# Autodesk Inventor assembly: Assembly Rack_4
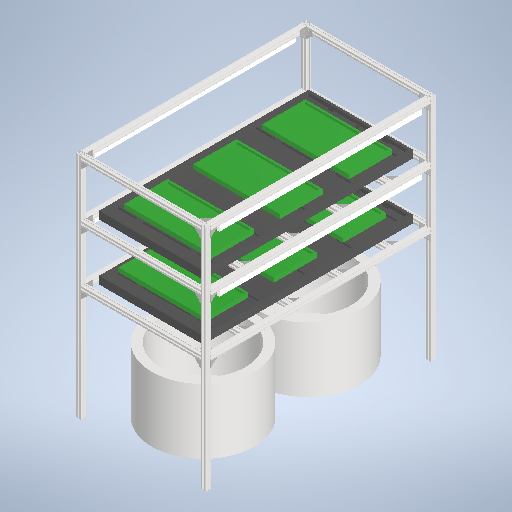
[picture p0: Inventor's stored thumbnail of the model, 512x512]
Saved by Autodesk Inventor 2025 (Build 290162000, 162)
## iProperties
Created: 2024-07-22
Part Number: Assembly Rack_4
Document SubType Name: Assembly
Designer: User
Author: User
## Documents named in this file (9)
- C:\Users\User\OneDrive\Documents\FYP\Inventor_Designs\Rack\Assembly Rack_4.iam
- C:\Users\User\OneDrive\Documents\FYP\Inventor_Designs\Rack\Water system 2.0\Metal_Profile 70cm.ipt
- C:\Users\User\OneDrive\Documents\FYP\Inventor_Designs\Rack\Light tube 118.4cm.ipt
- C:\Users\User\OneDrive\Documents\FYP\Inventor_Designs\Rack\flood tray.ipt
- C:\Users\User\OneDrive\Documents\FYP\Inventor_Designs\Rack\Tub.ipt
- C:\Users\User\OneDrive\Documents\FYP\Inventor_Designs\Platform\Potting Tray.ipt
- C:\Users\User\OneDrive\Documents\FYP\Inventor_Designs\Metal Profile\Metal Profile 129 cm.ipt
- C:\Users\User\OneDrive\Documents\FYP\Inventor_Designs\Metal Profile\Metal Profile 134 cm.ipt
- C:\Users\User\OneDrive\Documents\FYP\Inventor_Designs\L Bracket\L Angle Bracket 30x30.ipt
## Components (90 placed, 8 different names)
1. Metal_Profile 70cm:1 — Flush:89, Flush:103, Mate:83, Flush:106, Mate:96, Flush:141, Mate:140, Flush:142, Mate:146, Flush:145, Mate:158, Flush:170, Mate:195
2. Metal_Profile 70cm:2 — Flush:107, Flush:108, Mate:85, Mate:99, Mate:129, Mate:152, Mate:188, Flush:166, Mate:217
3. Metal_Profile 70cm:3 — Flush:104, Mate:84, Flush:105, Mate:105, Mate:138, Mate:144, Mate:156, Flush:169, Mate:193
4. Metal_Profile 70cm:4 — Flush:109, Flush:110, Mate:86, Mate:109, Mate:118, Flush:128, Mate:150, Mate:186, Flush:165, Mate:214
5. Metal_Profile 70cm:5 — Flush:78, Mate:70, Flush:79, Mate:71, Flush:80, Flush:82, Mate:72, Flush:83, Flush:84, Flush:85, Flush:97, Mate:114, Mate:142, Mate:154, Flush:167, Mate:191, Flush:168
6. Metal_Profile 70cm:6 — Mate:74, Mate:77, Mate:82, Flush:99, Mate:117, Mate:148, Flush:146, Mate:184, Flush:164, Mate:213
7. Light tube 118.4cm:1 — Flush:113, Mate:91, Mate:92
8. Light tube 118.4cm:2 — Mate:89, Flush:112, Mate:90
9. Light tube 118.4cm:3 — Flush:111, Mate:87, Mate:88
10. Light tube 118.4cm:4 — Mate:93, Flush:114, Mate:94
11. flood tray:1 — Mate:113
12. Tub:1
13. Potting Tray:1
14. Potting Tray:2
15. Potting Tray:3
16. Potting Tray:4
17. Potting Tray:5
18. Potting Tray:6
19. Metal_Profile 70cm:9 — Mate:95, Flush:115, Mate:96, Mate:101, Mate:112, Mate:136, Flush:140, Flush:176, Mate:205
20. Metal_Profile 70cm:14 — Flush:116, Mate:98, Mate:99, Mate:103, Mate:130, Flush:179, Mate:211
21. flood tray:2 — Mate:112, Flush:123
22. Metal Profile 129 cm:2 — Mate:70, Flush:79, Flush:81, Flush:87, Mate:75, Mate:82, Flush:113, Mate:92, Flush:124, Mate:115, Mate:116, Flush:126, Mate:176, Flush:160, Mate:178, Flush:161
23. Metal Profile 129 cm:4 — Mate:81, Flush:96, Flush:102, Flush:105, Flush:114, Mate:94, Flush:127, Mate:119, Mate:120, Flush:129, Flush:130, Mate:123, Flush:131, Flush:132, Mate:125, Mate:127, Mate:139, Mate:174, Flush:159, Mate:180, Flush:162
24. Metal Profile 129 cm:5 — Flush:78, Flush:85, Flush:86, Mate:73, Flush:88, Mate:76, Flush:98, Flush:100, Flush:111, Mate:88, Mate:160, Mate:170, Flush:157, Mate:190, Mate:212, Flush:180
25. Metal Profile 129 cm:6 — Mate:79, Flush:92, Flush:102, Flush:106, Flush:135, Mate:128, Mate:131, Flush:136, Mate:133, Mate:134, Flush:139, Mate:137, Mate:141, Mate:172, Flush:158, Mate:182, Flush:163
26. Metal Profile 134 cm:1 — Flush:82, Mate:72, Flush:83, Flush:84, Flush:86, Mate:73, Mate:78, Flush:90, Mate:80, Flush:93, Mate:83, Flush:104, Mate:84, Mate:87, Mate:90, Flush:149, Mate:155, Flush:150, Mate:157, Flush:151, Mate:159, Flush:152, Mate:161, Flush:153, Mate:163, Flush:154, Mate:164
27. Metal Profile 134 cm:2 — Mate:71, Flush:80, Flush:81, Mate:79, Flush:92, Mate:81, Flush:96, Flush:97, Flush:103, Mate:91, Mate:93, Flush:143, Mate:143, Flush:144, Mate:145, Mate:147, Mate:179, Mate:181, Mate:183
28. Metal Profile 134 cm:3 — Flush:88, Mate:76, Mate:77, Flush:98, Flush:99, Flush:108, Mate:85, Flush:110, Mate:86, Flush:155, Mate:167, Flush:156, Mate:169, Mate:171, Mate:185, Mate:187, Mate:189
29. Metal Profile 134 cm:4 — Flush:87, Mate:74, Mate:75, Mate:149, Flush:147, Mate:151, Flush:148, Mate:153, Mate:173, Mate:175, Mate:177
30. Metal Profile 129 cm:7 — Mate:80, Flush:93, Flush:100, Flush:101, Flush:109, Mate:89, Flush:112, Mate:104, Flush:119, Mate:106, Flush:120, Mate:108, Flush:121, Mate:110, Flush:122, Mate:162, Mate:168, Mate:192, Mate:196, Mate:198, Mate:200, Mate:202, Flush:181, Mate:215
31. Metal Profile 129 cm:8 — Flush:89, Mate:78, Flush:90, Flush:101, Flush:107, Mate:95, Flush:115, Flush:116, Mate:98, Mate:100, Flush:117, Mate:102, Flush:118, Flush:123, Mate:165, Mate:166, Mate:194, Mate:204, Mate:206, Mate:208, Flush:178, Mate:210, Mate:216, Flush:182
32. Metal_Profile 70cm:15 — Mate:106, Flush:120, Mate:107, Mate:113, Mate:124, Flush:172, Mate:199, Flush:173
33. Metal_Profile 70cm:16 — Mate:104, Flush:119, Mate:105, Mate:107, Mate:126, Flush:134, Flush:171, Mate:197
34. Metal_Profile 70cm:17 — Mate:102, Flush:118, Mate:103, Mate:132, Flush:137, Mate:209
35. Metal_Profile 70cm:18 — Mate:100, Flush:117, Mate:101, Flush:138, Mate:135, Flush:177, Mate:207
36. Metal_Profile 70cm:19 — Mate:110, Flush:122, Mate:111, Mate:122, Flush:174, Mate:201
37. Metal_Profile 70cm:21 — Mate:108, Flush:121, Mate:109, Mate:111, Mate:121, Flush:175, Mate:203
38. L Angle Bracket 30x30:24 — Flush:124, Mate:114, Mate:115
39. L Angle Bracket 30x30:25 — Mate:122, Mate:123, Flush:131
40. L Angle Bracket 30x30:26 — Mate:126, Flush:134, Mate:127
41. L Angle Bracket 30x30:30 — Mate:118, Flush:128, Mate:119
42. L Angle Bracket 30x30:31 — Flush:127, Mate:120, Flush:129, Mate:121
43. L Angle Bracket 30x30:32 — Mate:116, Flush:126, Mate:117
44. L Angle Bracket 30x30:33 — Flush:130, Flush:132, Mate:124, Mate:125
45. L Angle Bracket 30x30:34 — Mate:132, Flush:137, Mate:133
46. L Angle Bracket 30x30:35 — Mate:136, Flush:140, Mate:137
47. L Angle Bracket 30x30:36 — Flush:135, Mate:128, Mate:129
48. L Angle Bracket 30x30:37 — Flush:138, Mate:134, Mate:135, Flush:139
49. L Angle Bracket 30x30:39 — Mate:130, Mate:131, Flush:136
50. L Angle Bracket 30x30:40 — Mate:138, Mate:139
51. L Angle Bracket 30x30:42 — Flush:141, Mate:140, Flush:142, Mate:141
52. L Angle Bracket 30x30:46 — Mate:142, Flush:143, Mate:143
53. L Angle Bracket 30x30:47 — Mate:144, Flush:144, Mate:145
54. L Angle Bracket 30x30:48 — Mate:156, Flush:150, Mate:157
55. L Angle Bracket 30x30:49 — Mate:160, Flush:152, Mate:161
56. L Angle Bracket 30x30:50 — Mate:150, Flush:147, Mate:151
57. L Angle Bracket 30x30:51 — Flush:154, Mate:164, Mate:165
58. L Angle Bracket 30x30:52 — Flush:153, Mate:162, Mate:163
59. L Angle Bracket 30x30:53 — Mate:152, Flush:148, Mate:153
60. L Angle Bracket 30x30:54 — Mate:148, Flush:146, Mate:149
61. L Angle Bracket 30x30:55 — Mate:154, Flush:149, Mate:155
62. L Angle Bracket 30x30:56 — Mate:158, Flush:151, Mate:159
63. L Angle Bracket 30x30:57 — Mate:146, Flush:145, Mate:147
64. L Angle Bracket 30x30:58 — Mate:170, Flush:157, Mate:171
65. L Angle Bracket 30x30:59 — Flush:156, Mate:168, Mate:169
66. L Angle Bracket 30x30:60 — Flush:155, Mate:166, Mate:167
67. L Angle Bracket 30x30:61 — Mate:172, Flush:158, Mate:173
68. L Angle Bracket 30x30:62 — Mate:174, Flush:159, Mate:175
69. L Angle Bracket 30x30:63 — Mate:176, Flush:160, Mate:177
70. L Angle Bracket 30x30:64 — Mate:182, Mate:183, Flush:163
71. L Angle Bracket 30x30:65 — Mate:178, Mate:179, Flush:161
72. L Angle Bracket 30x30:66 — Mate:180, Mate:181, Flush:162
73. L Angle Bracket 30x30:67 — Mate:184, Flush:164, Mate:185
74. L Angle Bracket 30x30:68 — Mate:186, Mate:187, Flush:165
75. L Angle Bracket 30x30:69 — Mate:188, Flush:166, Mate:189
76. L Angle Bracket 30x30:70 — Flush:169, Mate:192, Mate:193
77. L Angle Bracket 30x30:71 — Flush:167, Mate:190, Mate:191, Flush:168
78. L Angle Bracket 30x30:72 — Flush:170, Mate:194, Mate:195
79. L Angle Bracket 30x30:73 — Flush:177, Mate:206, Mate:207
80. L Angle Bracket 30x30:74 — Flush:175, Mate:202, Mate:203
81. L Angle Bracket 30x30:75 — Flush:176, Mate:204, Mate:205
82. L Angle Bracket 30x30:76 — Flush:171, Mate:196, Mate:197
83. L Angle Bracket 30x30:77 — Flush:179, Mate:210, Mate:211
84. L Angle Bracket 30x30:78 — Mate:208, Flush:178, Mate:209
85. L Angle Bracket 30x30:79 — Mate:198, Mate:199, Flush:173
86. L Angle Bracket 30x30:80 — Flush:172, Flush:174, Mate:200, Mate:201
87. L Angle Bracket 30x30:82 — Flush:181, Mate:214, Mate:215
88. L Angle Bracket 30x30:83 — Mate:212, Flush:180, Mate:213
89. L Angle Bracket 30x30:84 — Mate:216, Flush:182, Mate:217
90. Tub:2
## Relationships (262: Mate 159, Flush 103)
- [Flush] (60 mm): Metal_Profile 70cm:3 ↔ flood tray:1
- [Mate]: flood tray:1 ↔ Potting Tray:3
- [Mate]: flood tray:1 ↔ Potting Tray:1
- [Mate]: flood tray:1 ↔ Potting Tray:2
- [Mate] (30 mm): flood tray:1 ↔ Potting Tray:3
- [Mate] (50 mm): flood tray:1 ↔ Potting Tray:3
- [Mate] (30 mm): flood tray:1 ↔ Potting Tray:1
- [Mate] (150 mm): Potting Tray:1 ↔ Potting Tray:3
- [Mate] (30 mm): flood tray:1 ↔ Potting Tray:2
- [Mate] (150 mm): Potting Tray:1 ↔ Potting Tray:2
- [Mate] (150 mm): Potting Tray:4 ↔ Potting Tray:5
- [Mate] (150 mm): Potting Tray:5 ↔ Potting Tray:6
- [Mate]: Metal_Profile 70cm:14 ↔ flood tray:2
- [Flush]: flood tray:1 ↔ flood tray:2
- [Flush]: flood tray:1 ↔ flood tray:2
- Flush:78: Metal_Profile 70cm:5 ↔ Metal Profile 129 cm:5
- Mate:70: Metal_Profile 70cm:5 ↔ Metal Profile 129 cm:2
- Flush:79: Metal_Profile 70cm:5 ↔ Metal Profile 129 cm:2
- Mate:71: Metal_Profile 70cm:5 ↔ Metal Profile 134 cm:2
- Flush:80: Metal_Profile 70cm:5 ↔ Metal Profile 134 cm:2
- Flush:81: Metal Profile 129 cm:2 ↔ Metal Profile 134 cm:2
- Flush:82: Metal_Profile 70cm:5 ↔ Metal Profile 134 cm:1
- Mate:72: Metal_Profile 70cm:5 ↔ Metal Profile 134 cm:1
- Flush:83: Metal_Profile 70cm:5 ↔ Metal Profile 134 cm:1
- Flush:84: Metal_Profile 70cm:5 ↔ Metal Profile 134 cm:1
- Flush:85: Metal_Profile 70cm:5 ↔ Metal Profile 129 cm:5
- Flush:86: Metal Profile 129 cm:5 ↔ Metal Profile 134 cm:1
- Mate:73: Metal Profile 129 cm:5 ↔ Metal Profile 134 cm:1
- Flush:87: Metal Profile 129 cm:2 ↔ Metal Profile 134 cm:4
- Mate:74: Metal_Profile 70cm:6 ↔ Metal Profile 134 cm:4
- Mate:75: Metal Profile 129 cm:2 ↔ Metal Profile 134 cm:4
- Flush:88: Metal Profile 129 cm:5 ↔ Metal Profile 134 cm:3
- Mate:76: Metal Profile 129 cm:5 ↔ Metal Profile 134 cm:3
- Mate:77: Metal_Profile 70cm:6 ↔ Metal Profile 134 cm:3
- Flush:89: Metal_Profile 70cm:1 ↔ Metal Profile 129 cm:8
- Mate:78: Metal Profile 134 cm:1 ↔ Metal Profile 129 cm:8
- Flush:90: Metal Profile 134 cm:1 ↔ Metal Profile 129 cm:8
- Mate:79: Metal Profile 129 cm:6 ↔ Metal Profile 134 cm:2
- Flush:92: Metal Profile 129 cm:6 ↔ Metal Profile 134 cm:2
- Mate:80: Metal Profile 134 cm:1 ↔ Metal Profile 129 cm:7
- Flush:93: Metal Profile 134 cm:1 ↔ Metal Profile 129 cm:7
- Mate:81: Metal Profile 129 cm:4 ↔ Metal Profile 134 cm:2
- Flush:96: Metal Profile 129 cm:4 ↔ Metal Profile 134 cm:2
- Flush:97: Metal_Profile 70cm:5 ↔ Metal Profile 134 cm:2
- Mate:82: Metal_Profile 70cm:6 ↔ Metal Profile 129 cm:2
- Flush:98: Metal Profile 129 cm:5 ↔ Metal Profile 134 cm:3
- Flush:99: Metal_Profile 70cm:6 ↔ Metal Profile 134 cm:3
- Flush:100 (330 mm): Metal Profile 129 cm:5 ↔ Metal Profile 129 cm:7
- Flush:101 (330 mm): Metal Profile 129 cm:7 ↔ Metal Profile 129 cm:8
- Flush:102 (330 mm): Metal Profile 129 cm:4 ↔ Metal Profile 129 cm:6
- Flush:103: Metal_Profile 70cm:1 ↔ Metal Profile 134 cm:2
- Mate:83: Metal_Profile 70cm:1 ↔ Metal Profile 134 cm:1
- Flush:104: Metal_Profile 70cm:3 ↔ Metal Profile 134 cm:1
- Mate:84: Metal_Profile 70cm:3 ↔ Metal Profile 134 cm:1
- Flush:105: Metal_Profile 70cm:3 ↔ Metal Profile 129 cm:4
- Flush:106: Metal_Profile 70cm:1 ↔ Metal Profile 129 cm:6
- Flush:107: Metal_Profile 70cm:2 ↔ Metal Profile 129 cm:8
- Flush:108: Metal_Profile 70cm:2 ↔ Metal Profile 134 cm:3
- Mate:85: Metal_Profile 70cm:2 ↔ Metal Profile 134 cm:3
- Flush:109: Metal_Profile 70cm:4 ↔ Metal Profile 129 cm:7
- Flush:110: Metal_Profile 70cm:4 ↔ Metal Profile 134 cm:3
- Mate:86: Metal_Profile 70cm:4 ↔ Metal Profile 134 cm:3
- Flush:111: Light tube 118.4cm:3 ↔ Metal Profile 129 cm:5
- Mate:87 (50 mm): Light tube 118.4cm:3 ↔ Metal Profile 134 cm:1
- Mate:88: Light tube 118.4cm:3 ↔ Metal Profile 129 cm:5
- Mate:89: Light tube 118.4cm:2 ↔ Metal Profile 129 cm:7
- Flush:112: Light tube 118.4cm:2 ↔ Metal Profile 129 cm:7
- Mate:90 (50 mm): Light tube 118.4cm:2 ↔ Metal Profile 134 cm:1
- Flush:113: Light tube 118.4cm:1 ↔ Metal Profile 129 cm:2
- Mate:91 (50 mm): Light tube 118.4cm:1 ↔ Metal Profile 134 cm:2
- Mate:92: Light tube 118.4cm:1 ↔ Metal Profile 129 cm:2
- Mate:93 (50 mm): Light tube 118.4cm:4 ↔ Metal Profile 134 cm:2
- Flush:114: Light tube 118.4cm:4 ↔ Metal Profile 129 cm:4
- Mate:94: Light tube 118.4cm:4 ↔ Metal Profile 129 cm:4
- Mate:95: Metal_Profile 70cm:9 ↔ Metal Profile 129 cm:8
- Flush:115: Metal_Profile 70cm:9 ↔ Metal Profile 129 cm:8
- Mate:96 (200 mm): Metal_Profile 70cm:1 ↔ Metal_Profile 70cm:9
- Flush:116: Metal_Profile 70cm:14 ↔ Metal Profile 129 cm:8
- Mate:98: Metal_Profile 70cm:14 ↔ Metal Profile 129 cm:8
- Mate:99 (200 mm): Metal_Profile 70cm:2 ↔ Metal_Profile 70cm:14
- Mate:100: Metal Profile 129 cm:8 ↔ Metal_Profile 70cm:18
- Flush:117: Metal Profile 129 cm:8 ↔ Metal_Profile 70cm:18
- Mate:101 (255 mm): Metal_Profile 70cm:9 ↔ Metal_Profile 70cm:18
- Mate:102: Metal Profile 129 cm:8 ↔ Metal_Profile 70cm:17
- Flush:118: Metal Profile 129 cm:8 ↔ Metal_Profile 70cm:17
- Mate:103 (255 mm): Metal_Profile 70cm:14 ↔ Metal_Profile 70cm:17
- Mate:104: Metal Profile 129 cm:7 ↔ Metal_Profile 70cm:16
- Flush:119: Metal Profile 129 cm:7 ↔ Metal_Profile 70cm:16
- Mate:105 (200 mm): Metal_Profile 70cm:3 ↔ Metal_Profile 70cm:16
- Mate:106: Metal Profile 129 cm:7 ↔ Metal_Profile 70cm:15
- Flush:120: Metal Profile 129 cm:7 ↔ Metal_Profile 70cm:15
- Mate:107 (255 mm): Metal_Profile 70cm:15 ↔ Metal_Profile 70cm:16
- Mate:108: Metal Profile 129 cm:7 ↔ Metal_Profile 70cm:21
- Flush:121: Metal Profile 129 cm:7 ↔ Metal_Profile 70cm:21
- Mate:109 (200 mm): Metal_Profile 70cm:4 ↔ Metal_Profile 70cm:21
- Mate:110: Metal Profile 129 cm:7 ↔ Metal_Profile 70cm:19
- Flush:122: Metal Profile 129 cm:7 ↔ Metal_Profile 70cm:19
- Mate:111 (255 mm): Metal_Profile 70cm:19 ↔ Metal_Profile 70cm:21
- Mate:112: Metal_Profile 70cm:9 ↔ flood tray:2
- Flush:123 (75 mm): flood tray:2 ↔ Metal Profile 129 cm:8
- Mate:113: flood tray:1 ↔ Metal_Profile 70cm:15
- Flush:124: Metal Profile 129 cm:2 ↔ L Angle Bracket 30x30:24
- Mate:114: Metal_Profile 70cm:5 ↔ L Angle Bracket 30x30:24
- Mate:115: Metal Profile 129 cm:2 ↔ L Angle Bracket 30x30:24
- Mate:116: Metal Profile 129 cm:2 ↔ L Angle Bracket 30x30:32
- Flush:126: Metal Profile 129 cm:2 ↔ L Angle Bracket 30x30:32
- Mate:117: Metal_Profile 70cm:6 ↔ L Angle Bracket 30x30:32
- Flush:127: Metal Profile 129 cm:4 ↔ L Angle Bracket 30x30:31
- Mate:118: Metal_Profile 70cm:4 ↔ L Angle Bracket 30x30:30
- Flush:128: Metal_Profile 70cm:4 ↔ L Angle Bracket 30x30:30
- Mate:119: Metal Profile 129 cm:4 ↔ L Angle Bracket 30x30:30
- Mate:120: Metal Profile 129 cm:4 ↔ L Angle Bracket 30x30:31
- Flush:129: Metal Profile 129 cm:4 ↔ L Angle Bracket 30x30:31
- Mate:121: Metal_Profile 70cm:21 ↔ L Angle Bracket 30x30:31
- Flush:130: Metal Profile 129 cm:4 ↔ L Angle Bracket 30x30:33
- Mate:122: Metal_Profile 70cm:19 ↔ L Angle Bracket 30x30:25
- Mate:123: Metal Profile 129 cm:4 ↔ L Angle Bracket 30x30:25
- Flush:131: Metal Profile 129 cm:4 ↔ L Angle Bracket 30x30:25
- Flush:132: Metal Profile 129 cm:4 ↔ L Angle Bracket 30x30:33
- Mate:124: Metal_Profile 70cm:15 ↔ L Angle Bracket 30x30:33
- Mate:125: Metal Profile 129 cm:4 ↔ L Angle Bracket 30x30:33
- Mate:126: Metal_Profile 70cm:16 ↔ L Angle Bracket 30x30:26
- Flush:134: Metal_Profile 70cm:16 ↔ L Angle Bracket 30x30:26
- Mate:127: Metal Profile 129 cm:4 ↔ L Angle Bracket 30x30:26
- Flush:135: Metal Profile 129 cm:6 ↔ L Angle Bracket 30x30:36
- Mate:128: Metal Profile 129 cm:6 ↔ L Angle Bracket 30x30:36
- Mate:129: Metal_Profile 70cm:2 ↔ L Angle Bracket 30x30:36
- Mate:130: Metal_Profile 70cm:14 ↔ L Angle Bracket 30x30:39
- Mate:131: Metal Profile 129 cm:6 ↔ L Angle Bracket 30x30:39
- Flush:136: Metal Profile 129 cm:6 ↔ L Angle Bracket 30x30:39
- Mate:132: Metal_Profile 70cm:17 ↔ L Angle Bracket 30x30:34
- Flush:137: Metal_Profile 70cm:17 ↔ L Angle Bracket 30x30:34
- Mate:133: Metal Profile 129 cm:6 ↔ L Angle Bracket 30x30:34
- Flush:138: Metal_Profile 70cm:18 ↔ L Angle Bracket 30x30:37
- Mate:134: Metal Profile 129 cm:6 ↔ L Angle Bracket 30x30:37
- Mate:135: Metal_Profile 70cm:18 ↔ L Angle Bracket 30x30:37
- Flush:139: Metal Profile 129 cm:6 ↔ L Angle Bracket 30x30:37
- Mate:136: Metal_Profile 70cm:9 ↔ L Angle Bracket 30x30:35
- Flush:140: Metal_Profile 70cm:9 ↔ L Angle Bracket 30x30:35
- Mate:137: Metal Profile 129 cm:6 ↔ L Angle Bracket 30x30:35
- Mate:138: Metal_Profile 70cm:3 ↔ L Angle Bracket 30x30:40
- Mate:139: Metal Profile 129 cm:4 ↔ L Angle Bracket 30x30:40
- Flush:141: Metal_Profile 70cm:1 ↔ L Angle Bracket 30x30:42
- Mate:140: Metal_Profile 70cm:1 ↔ L Angle Bracket 30x30:42
- Flush:142: Metal_Profile 70cm:1 ↔ L Angle Bracket 30x30:42
- Mate:141: Metal Profile 129 cm:6 ↔ L Angle Bracket 30x30:42
- Mate:142: Metal_Profile 70cm:5 ↔ L Angle Bracket 30x30:46
- Flush:143: Metal Profile 134 cm:2 ↔ L Angle Bracket 30x30:46
- Mate:143: Metal Profile 134 cm:2 ↔ L Angle Bracket 30x30:46
- Mate:144: Metal_Profile 70cm:3 ↔ L Angle Bracket 30x30:47
- Flush:144: Metal Profile 134 cm:2 ↔ L Angle Bracket 30x30:47
- Mate:145: Metal Profile 134 cm:2 ↔ L Angle Bracket 30x30:47
- Mate:146: Metal_Profile 70cm:1 ↔ L Angle Bracket 30x30:57
- Flush:145: Metal_Profile 70cm:1 ↔ L Angle Bracket 30x30:57
- Mate:147: Metal Profile 134 cm:2 ↔ L Angle Bracket 30x30:57
- Mate:148: Metal_Profile 70cm:6 ↔ L Angle Bracket 30x30:54
- Flush:146: Metal_Profile 70cm:6 ↔ L Angle Bracket 30x30:54
- Mate:149: Metal Profile 134 cm:4 ↔ L Angle Bracket 30x30:54
- Mate:150: Metal_Profile 70cm:4 ↔ L Angle Bracket 30x30:50
- Flush:147: Metal Profile 134 cm:4 ↔ L Angle Bracket 30x30:50
- Mate:151: Metal Profile 134 cm:4 ↔ L Angle Bracket 30x30:50
- Mate:152: Metal_Profile 70cm:2 ↔ L Angle Bracket 30x30:53
- Flush:148: Metal Profile 134 cm:4 ↔ L Angle Bracket 30x30:53
- Mate:153: Metal Profile 134 cm:4 ↔ L Angle Bracket 30x30:53
- Mate:154: Metal_Profile 70cm:5 ↔ L Angle Bracket 30x30:55
- Flush:149: Metal Profile 134 cm:1 ↔ L Angle Bracket 30x30:55
- Mate:155: Metal Profile 134 cm:1 ↔ L Angle Bracket 30x30:55
- Mate:156: Metal_Profile 70cm:3 ↔ L Angle Bracket 30x30:48
- Flush:150: Metal Profile 134 cm:1 ↔ L Angle Bracket 30x30:48
- Mate:157: Metal Profile 134 cm:1 ↔ L Angle Bracket 30x30:48
- Mate:158: Metal_Profile 70cm:1 ↔ L Angle Bracket 30x30:56
- Flush:151: Metal Profile 134 cm:1 ↔ L Angle Bracket 30x30:56
- Mate:159: Metal Profile 134 cm:1 ↔ L Angle Bracket 30x30:56
- Mate:160: Metal Profile 129 cm:5 ↔ L Angle Bracket 30x30:49
- Flush:152: Metal Profile 134 cm:1 ↔ L Angle Bracket 30x30:49
- Mate:161: Metal Profile 134 cm:1 ↔ L Angle Bracket 30x30:49
- Flush:153: Metal Profile 134 cm:1 ↔ L Angle Bracket 30x30:52
- Mate:162: Metal Profile 129 cm:7 ↔ L Angle Bracket 30x30:52
- Mate:163: Metal Profile 134 cm:1 ↔ L Angle Bracket 30x30:52
- Flush:154: Metal Profile 134 cm:1 ↔ L Angle Bracket 30x30:51
- Mate:164: Metal Profile 134 cm:1 ↔ L Angle Bracket 30x30:51
- Mate:165: Metal Profile 129 cm:8 ↔ L Angle Bracket 30x30:51
- Flush:155: Metal Profile 134 cm:3 ↔ L Angle Bracket 30x30:60
- Mate:166: Metal Profile 129 cm:8 ↔ L Angle Bracket 30x30:60
- Mate:167: Metal Profile 134 cm:3 ↔ L Angle Bracket 30x30:60
- Flush:156: Metal Profile 134 cm:3 ↔ L Angle Bracket 30x30:59
- Mate:168: Metal Profile 129 cm:7 ↔ L Angle Bracket 30x30:59
- Mate:169: Metal Profile 134 cm:3 ↔ L Angle Bracket 30x30:59
- Mate:170: Metal Profile 129 cm:5 ↔ L Angle Bracket 30x30:58
- Flush:157: Metal Profile 129 cm:5 ↔ L Angle Bracket 30x30:58
- Mate:171: Metal Profile 134 cm:3 ↔ L Angle Bracket 30x30:58
- Mate:172: Metal Profile 129 cm:6 ↔ L Angle Bracket 30x30:61
- Flush:158: Metal Profile 129 cm:6 ↔ L Angle Bracket 30x30:61
- Mate:173: Metal Profile 134 cm:4 ↔ L Angle Bracket 30x30:61
- Mate:174: Metal Profile 129 cm:4 ↔ L Angle Bracket 30x30:62
- Flush:159: Metal Profile 129 cm:4 ↔ L Angle Bracket 30x30:62
- Mate:175: Metal Profile 134 cm:4 ↔ L Angle Bracket 30x30:62
- Mate:176: Metal Profile 129 cm:2 ↔ L Angle Bracket 30x30:63
- Flush:160: Metal Profile 129 cm:2 ↔ L Angle Bracket 30x30:63
- Mate:177: Metal Profile 134 cm:4 ↔ L Angle Bracket 30x30:63
- Mate:178: Metal Profile 129 cm:2 ↔ L Angle Bracket 30x30:65
- Mate:179: Metal Profile 134 cm:2 ↔ L Angle Bracket 30x30:65
- Flush:161: Metal Profile 129 cm:2 ↔ L Angle Bracket 30x30:65
- Mate:180: Metal Profile 129 cm:4 ↔ L Angle Bracket 30x30:66
- Mate:181: Metal Profile 134 cm:2 ↔ L Angle Bracket 30x30:66
- Flush:162: Metal Profile 129 cm:4 ↔ L Angle Bracket 30x30:66
- Mate:182: Metal Profile 129 cm:6 ↔ L Angle Bracket 30x30:64
- Mate:183: Metal Profile 134 cm:2 ↔ L Angle Bracket 30x30:64
- Flush:163: Metal Profile 129 cm:6 ↔ L Angle Bracket 30x30:64
- Mate:184: Metal_Profile 70cm:6 ↔ L Angle Bracket 30x30:67
- Flush:164: Metal_Profile 70cm:6 ↔ L Angle Bracket 30x30:67
- Mate:185: Metal Profile 134 cm:3 ↔ L Angle Bracket 30x30:67
- Mate:186: Metal_Profile 70cm:4 ↔ L Angle Bracket 30x30:68
- Mate:187: Metal Profile 134 cm:3 ↔ L Angle Bracket 30x30:68
- Flush:165: Metal_Profile 70cm:4 ↔ L Angle Bracket 30x30:68
- Mate:188: Metal_Profile 70cm:2 ↔ L Angle Bracket 30x30:69
- Flush:166: Metal_Profile 70cm:2 ↔ L Angle Bracket 30x30:69
- Mate:189: Metal Profile 134 cm:3 ↔ L Angle Bracket 30x30:69
- Flush:167: Metal_Profile 70cm:5 ↔ L Angle Bracket 30x30:71
- Mate:190: Metal Profile 129 cm:5 ↔ L Angle Bracket 30x30:71
- Mate:191: Metal_Profile 70cm:5 ↔ L Angle Bracket 30x30:71
- Flush:168: Metal_Profile 70cm:5 ↔ L Angle Bracket 30x30:71
- Flush:169: Metal_Profile 70cm:3 ↔ L Angle Bracket 30x30:70
- Mate:192: Metal Profile 129 cm:7 ↔ L Angle Bracket 30x30:70
- Mate:193: Metal_Profile 70cm:3 ↔ L Angle Bracket 30x30:70
- Flush:170: Metal_Profile 70cm:1 ↔ L Angle Bracket 30x30:72
- Mate:194: Metal Profile 129 cm:8 ↔ L Angle Bracket 30x30:72
- Mate:195: Metal_Profile 70cm:1 ↔ L Angle Bracket 30x30:72
- Flush:171: Metal_Profile 70cm:16 ↔ L Angle Bracket 30x30:76
- Mate:196: Metal Profile 129 cm:7 ↔ L Angle Bracket 30x30:76
- Mate:197: Metal_Profile 70cm:16 ↔ L Angle Bracket 30x30:76
- Flush:172: Metal_Profile 70cm:15 ↔ L Angle Bracket 30x30:80
- Mate:198: Metal Profile 129 cm:7 ↔ L Angle Bracket 30x30:79
- Mate:199: Metal_Profile 70cm:15 ↔ L Angle Bracket 30x30:79
- Flush:173: Metal_Profile 70cm:15 ↔ L Angle Bracket 30x30:79
- Flush:174: Metal_Profile 70cm:19 ↔ L Angle Bracket 30x30:80
- Mate:200: Metal Profile 129 cm:7 ↔ L Angle Bracket 30x30:80
- Mate:201: Metal_Profile 70cm:19 ↔ L Angle Bracket 30x30:80
- Flush:175: Metal_Profile 70cm:21 ↔ L Angle Bracket 30x30:74
- Mate:202: Metal Profile 129 cm:7 ↔ L Angle Bracket 30x30:74
- Mate:203: Metal_Profile 70cm:21 ↔ L Angle Bracket 30x30:74
- Flush:176: Metal_Profile 70cm:9 ↔ L Angle Bracket 30x30:75
- Mate:204: Metal Profile 129 cm:8 ↔ L Angle Bracket 30x30:75
- Mate:205: Metal_Profile 70cm:9 ↔ L Angle Bracket 30x30:75
- Flush:177: Metal_Profile 70cm:18 ↔ L Angle Bracket 30x30:73
- Mate:206: Metal Profile 129 cm:8 ↔ L Angle Bracket 30x30:73
- Mate:207: Metal_Profile 70cm:18 ↔ L Angle Bracket 30x30:73
- Mate:208: Metal Profile 129 cm:8 ↔ L Angle Bracket 30x30:78
- Flush:178: Metal Profile 129 cm:8 ↔ L Angle Bracket 30x30:78
- Mate:209: Metal_Profile 70cm:17 ↔ L Angle Bracket 30x30:78
- Flush:179: Metal_Profile 70cm:14 ↔ L Angle Bracket 30x30:77
- Mate:210: Metal Profile 129 cm:8 ↔ L Angle Bracket 30x30:77
- Mate:211: Metal_Profile 70cm:14 ↔ L Angle Bracket 30x30:77
- Mate:212: Metal Profile 129 cm:5 ↔ L Angle Bracket 30x30:83
- Flush:180: Metal Profile 129 cm:5 ↔ L Angle Bracket 30x30:83
- Mate:213: Metal_Profile 70cm:6 ↔ L Angle Bracket 30x30:83
- Flush:181: Metal Profile 129 cm:7 ↔ L Angle Bracket 30x30:82
- Mate:214: Metal_Profile 70cm:4 ↔ L Angle Bracket 30x30:82
- Mate:215: Metal Profile 129 cm:7 ↔ L Angle Bracket 30x30:82
- Mate:216: Metal Profile 129 cm:8 ↔ L Angle Bracket 30x30:84
- Flush:182: Metal Profile 129 cm:8 ↔ L Angle Bracket 30x30:84
- Mate:217: Metal_Profile 70cm:2 ↔ L Angle Bracket 30x30:84
